# Autodesk Inventor assembly: 平行サスシャフト4
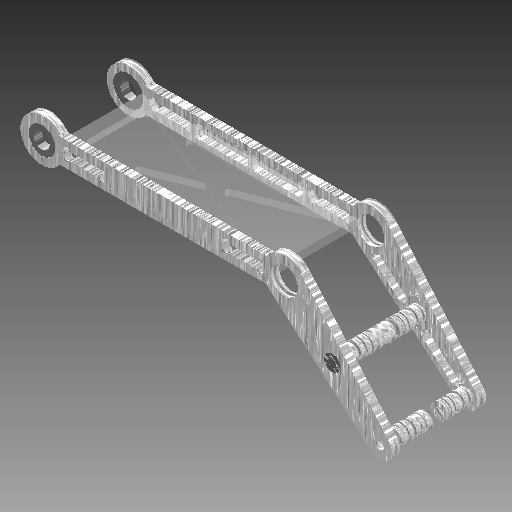
[picture p0: Inventor's stored thumbnail of the model, 512x512]
Saved by Autodesk Inventor 2020 (Build 240168000, 168)
## iProperties
Created: 2019-09-03
Part Number: 平行サスシャフト4
Document SubType Name: Assembly
Designer: 雪村
Mass: 29.696 g
Surface Area: 181.776 cm^2
Volume: 12.3815 cm^3
Density: 2.39841 g/cm^3
Author: 雪村
## Documents named in this file (10)
- C:\Users\white\Documents\SRDC\SRDC\Inventor_2017\2018年機体\2020年4年機体\平行サスシャフト4.iam
- C:\Users\white\Documents\SRDC\SRDC\Inventor_2017\2018年機体\2020年4年機体\平行サスシャフト3.ipt
- C:\Users\white\Documents\SRDC\SRDC\Inventor_2017\2018年機体\2020年4年機体\平行サス板4.ipt
- C:\Users\white\Documents\SRDC\SRDC\Inventor_2017\2018年機体\2020年4年機体\平行サスシャフト3_MIR.ipt
- C:\Users\white\Documents\SRDC\SRDC\Inventor_2017\2018年機体\パーツ\スペーサーm3,30.ipt
- C:\Users\white\Documents\SRDC\SRDC\Inventor_2017\2018年機体\パーツ\ネジ鍋m3,08.ipt
- C:\Users\white\Documents\SRDC\SRDC\Inventor_2017\2018年機体\パーツ\ネジ皿m3,08.ipt
- C:\Users\white\Documents\SRDC\SRDC\Inventor_2017\2018年機体\パーツ\ベアリングフランジ付き0610.3t.ipt
- C:\Users\white\Documents\SRDC\SRDC\Inventor_2017\2018年機体\パーツ\スペーサーm3,10.ipt
- C:\Users\white\Documents\SRDC\SRDC\Inventor_2017\2018年機体\パーツ\スペーサーm3,14.ipt
## Components (10 placed, 9 different names)
1. 平行サスシャフト3:1 — 挿入:1, 挿入:2, 挿入:4, 挿入:6, メイト:4, メイト:5, メイト:6
2. 平行サスシャフト3_MIR:1 — 挿入:3, 挿入:5, 挿入:7, メイト:1, メイト:2, メイト:3
3. スペーサーm3,30:1 — 挿入:1
4. ネジ鍋m3,08:1 — 挿入:2
5. ネジ皿m3,08:1 — 挿入:3
6. ベアリングフランジ付き0610.3t:1 — 挿入:4
7. ベアリングフランジ付き0610.3t:2 — 挿入:5
8. スペーサーm3,10:1 — 挿入:6
9. スペーサーm3,14:1 — 挿入:7
10. 平行サス板4:1 — メイト:1, メイト:2, メイト:3, メイト:4, メイト:5, メイト:6
## Relationships (13: Insert 7, Mate 6)
- 挿入:1 [Insert]: 平行サスシャフト3:1 ↔ スペーサーm3,30:1
- 挿入:2 [Insert]: 平行サスシャフト3:1 ↔ ネジ鍋m3,08:1
- 挿入:3 [Insert]: 平行サスシャフト3_MIR:1 ↔ ネジ皿m3,08:1
- 挿入:4 [Insert]: 平行サスシャフト3:1 ↔ ベアリングフランジ付き0610.3t:1
- 挿入:5 [Insert]: 平行サスシャフト3_MIR:1 ↔ ベアリングフランジ付き0610.3t:2
- 挿入:6 [Insert]: 平行サスシャフト3:1 ↔ スペーサーm3,10:1
- 挿入:7 [Insert]: 平行サスシャフト3_MIR:1 ↔ スペーサーm3,14:1
- メイト:1 [Mate]: 平行サスシャフト3_MIR:1 ↔ 平行サス板4:1
- メイト:2 [Mate]: 平行サスシャフト3_MIR:1 ↔ 平行サス板4:1
- メイト:3 [Mate]: 平行サスシャフト3_MIR:1 ↔ 平行サス板4:1
- メイト:4 [Mate]: 平行サスシャフト3:1 ↔ 平行サス板4:1
- メイト:5 [Mate]: 平行サスシャフト3:1 ↔ 平行サス板4:1
- メイト:6 [Mate]: 平行サスシャフト3:1 ↔ 平行サス板4:1
